# Autodesk Inventor assembly: zmotorblock
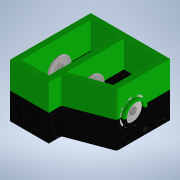
[picture p0: Inventor's stored thumbnail of the model, 180x180]
Saved by Autodesk Inventor 2020 (Build 240168000, 168)
## iProperties
Created: 2021-02-28
Part Number: zmotorblock
Document SubType Name: Assembly
Designer: AOB
Mass: 120.624 g
Surface Area: 407.974 cm^2
Volume: 82.7913 cm^3
Density: 1.45697 g/cm^3
Author: AOB
## Documents named in this file (4)
- C:\Users\marti\Documents\Inventor\ProjectBoron\ultimate boron\zmotorblock.iam
- C:\Users\marti\Documents\Inventor\ProjectBoron\ultimate boron\zmotorblockleft-half.ipt
- C:\Users\marti\Documents\Inventor\ProjectBoron\ultimate boron\zmotorblockright-half.ipt
- C:\Users\marti\Documents\Inventor\ProjectBoron\ultimate boron\flange-bearing.ipt
## Components (5 placed, 3 different names)
1. zmotorblockleft-half:1 — Flush:1, Flush:2, Flush:3, Rigid:1
2. zmotorblockright-half:1 — Flush:1, Flush:2, Flush:3, Mate:2, Mate:3, Mate:4, Mate:5, Rigid:1, Mate:6, Mate:7
3. flange-bearing:1 — Mate:2, Mate:3
4. flange-bearing:2 — Mate:4, Mate:5
5. flange-bearing:3 — Mate:6, Mate:7
## Relationships (10: Mate 6, Flush 3, WeldJoint 1)
- Flush:1: zmotorblockleft-half:1 ↔ zmotorblockright-half:1
- Flush:2: zmotorblockleft-half:1 ↔ zmotorblockright-half:1
- Flush:3: zmotorblockleft-half:1 ↔ zmotorblockright-half:1
- Mate:2: zmotorblockright-half:1 ↔ flange-bearing:1
- Mate:3: zmotorblockright-half:1 ↔ flange-bearing:1
- Mate:4: zmotorblockright-half:1 ↔ flange-bearing:2
- Mate:5: zmotorblockright-half:1 ↔ flange-bearing:2
- Rigid:1 [WeldJoint]: zmotorblockleft-half:1 ↔ zmotorblockright-half:1
- Mate:6: zmotorblockright-half:1 ↔ flange-bearing:3
- Mate:7: zmotorblockright-half:1 ↔ flange-bearing:3
